# Autodesk Inventor assembly: Ball Collection Mechanism
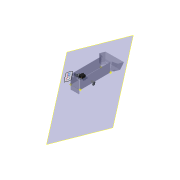
[picture p0: Inventor's stored thumbnail of the model, 180x180]
Saved by Autodesk Inventor 2015 SP1 (Build 190203100, 203)
## iProperties
Created: 2014-09-14
Part Number: Ball Collection Mechanism
Document SubType Name: Assembly
Designer: Family Room
Author: Family Room
## Documents named in this file (8)
- C:\Users\datenney\Documents\GitHub\CAD\2014_robotComplete\Ball Collection Mechanism.iam
- C:\Users\datenney\Documents\GitHub\CAD\2014_robotComplete\Imported Components\L bracket\L bracket.ipt
- C:\Users\datenney\Documents\GitHub\CAD\2014_robotComplete\Imported Components\Motor Hub\Motor Hub.ipt
- C:\Users\datenney\Documents\GitHub\CAD\2014_robotComplete\Imported Components\40 tooth Gear\40 tooth Gear.ipt
- C:\Users\datenney\Documents\GitHub\CAD\2014_robotComplete\Imported Components\singleservobracket\singleservobracket.ipt
- C:\Users\datenney\Documents\GitHub\CAD\2014_robotComplete\Imported Components\servo\servo.iam
- C:\Users\datenney\Documents\GitHub\CAD\2014_robotComplete\Ball Release.ipt
- C:\Users\datenney\Documents\GitHub\CAD\2014_robotComplete\Ball collector sheetmetal form.ipt
## Components (10 placed, 7 different names)
1. L bracket:1 — Mate:2, Flush:2, Flush:3, Insert:5, Insert:6, Flush:8
2. L bracket:2 — Mate:1, Flush:3, Insert:1, Flush:9, Symmetry:1
3. Ball collector sheetmetal form:1 — Mate:1, Mate:2, Flush:2, Mate:5, Flush:7, Flush:8, Flush:9, Symmetry:1
4. Motor Hub:1 — Insert:5
5. Motor Hub:2 — Insert:1
6. 40 tooth Gear:1 — Insert:6
7. singleservobracket:1 — Mate:3, Angle:1, Mate:4, Mate:5, Flush:7
8. servo:1 [sub-assembly] — Mate:3, Angle:1, Mate:4, Insert:4
9. L bracket:3 — Insert:4, Flush:5, Mate:6, Mate:7, Mate:8
10. Ball Release:1 — Mate:6, Mate:7, Mate:8
## Relationships (21: Mate 8, Flush 7, Insert 4, Angle 1, Symmetry 1)
- Mate:1: L bracket:2 ↔ Ball collector sheetmetal form:1
- [Flush]: L bracket:2 ↔ Ball collector sheetmetal form:1
- Mate:2: L bracket:1 ↔ Ball collector sheetmetal form:1
- Flush:2: L bracket:1 ↔ Ball collector sheetmetal form:1
- Flush:3: L bracket:1 ↔ L bracket:2
- Insert:1: L bracket:2 ↔ Motor Hub:2
- Mate:3: singleservobracket:1 ↔ servo:1
- Angle:1 (0 deg): singleservobracket:1 ↔ servo:1
- Mate:4: singleservobracket:1 ↔ servo:1
- Insert:4: servo:1 ↔ L bracket:3
- Mate:5: Ball collector sheetmetal form:1 ↔ singleservobracket:1
- Flush:5: L bracket:3
- Mate:6: L bracket:3 ↔ Ball Release:1
- Mate:7: L bracket:3 ↔ Ball Release:1
- Mate:8: L bracket:3 ↔ Ball Release:1
- Flush:7 (-2.286 mm): Ball collector sheetmetal form:1 ↔ singleservobracket:1
- Insert:5: L bracket:1 ↔ Motor Hub:1
- Insert:6: L bracket:1 ↔ 40 tooth Gear:1
- Flush:8 (139.7 mm): L bracket:1 ↔ Ball collector sheetmetal form:1
- Flush:9: L bracket:2 ↔ Ball collector sheetmetal form:1
- Symmetry:1: L bracket:2 ↔ Ball collector sheetmetal form:1
